# Autodesk Inventor assembly: LIVER SUBASSEMBLY
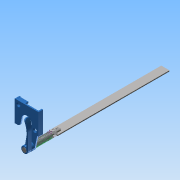
[picture p0: Inventor's stored thumbnail of the model, 180x180]
Saved by Autodesk Inventor 2014 SP1 (Build 180222100, 222)
## iProperties
Created: 2014-12-19
Part Number: LIVER SUBASSEMBLY
Document SubType Name: Assembly
Designer: Ebrahim
Author: Ebrahim
## Documents named in this file (8)
- D:\MY D OLD DRIVE\Ibrahim folder on Drlab216\2014-2015\BENCH VICE PACKED\Workspace\LIVER SUBASSEMBLY.iam
- D:\MY D OLD DRIVE\Ibrahim folder on Drlab216\2014-2015\BENCH VICE PACKED\Workspace\LIVER CAP.ipt
- D:\MY D OLD DRIVE\Ibrahim folder on Drlab216\2014-2015\BENCH VICE PACKED\Workspace\LIVER SHAFT.ipt
- D:\MY D OLD DRIVE\Ibrahim folder on Drlab216\2014-2015\BENCH VICE PACKED\Workspace\LIVER HANDLE.ipt
- D:\MY D OLD DRIVE\Ibrahim folder on Drlab216\2014-2015\BENCH VICE PACKED\Workspace\LIVER.ipt
- D:\MY D OLD DRIVE\Ibrahim folder on Drlab216\2014-2015\BENCH VICE PACKED\Workspace\SPRING NUT1.ipt
- D:\MY D OLD DRIVE\Ibrahim folder on Drlab216\2014-2015\BENCH VICE PACKED\Workspace\LIVER SUBASSEMBLY\Design Accelerator\Compress Spring1.iam
- D:\MY D OLD DRIVE\Ibrahim folder on Drlab216\2014-2015\BENCH VICE PACKED\Libraries\Content Center Files\en-US\ISO 2341 A(1)\ISO 2341 - A - 3 x 14ISO.ipt
## Components (7 placed, 7 different names)
1. LIVER CAP:1 — Insert:2, Flush:3, Flush:5
2. LIVER SHAFT:1 — Insert:1, Flush:1, Insert:3, Mate:4, Mate:7, Mate:9, Flush:4, Flush:5
3. LIVER HANDLE:1 — Insert:1, Insert:2, Flush:1
4. LIVER:1 — Insert:3, Mate:8, Flush:4, Mate:10, Mate:11
5. Compress Spring:1 [sub-assembly] — Flush:3, Mate:4
6. ISO 2341 A A - 3 x 14:1 — Mate:7, Mate:8
7. SPRING NUT1:1 — Mate:9, Mate:10, Mate:11
## Relationships (13: Mate 6, Flush 4, Insert 3)
- Insert:1 (1 mm): LIVER SHAFT:1 ↔ LIVER HANDLE:1
- Insert:2: LIVER CAP:1 ↔ LIVER HANDLE:1
- Flush:1: LIVER SHAFT:1 ↔ LIVER HANDLE:1
- Insert:3: LIVER SHAFT:1 ↔ LIVER:1
- Flush:3: LIVER CAP:1 ↔ Compress Spring:1
- Mate:4: LIVER SHAFT:1 ↔ Compress Spring:1
- Mate:7: LIVER SHAFT:1 ↔ ISO 2341 A A - 3 x 14:1
- Mate:8 (5 mm): LIVER:1 ↔ ISO 2341 A A - 3 x 14:1
- Mate:9: LIVER SHAFT:1 ↔ SPRING NUT1:1
- Flush:4 (-1.5 mm): LIVER SHAFT:1 ↔ LIVER:1
- Mate:10: LIVER:1 ↔ SPRING NUT1:1
- Mate:11: LIVER:1 ↔ SPRING NUT1:1
- Flush:5: LIVER CAP:1 ↔ LIVER SHAFT:1
